# Autodesk Inventor assembly: 15inOwl
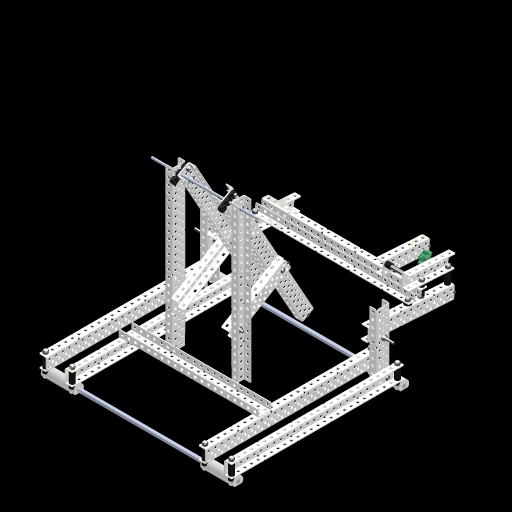
[picture p0: Inventor's stored thumbnail of the model, 512x512]
Saved by Autodesk Inventor 2024.1 (Build 281209000, 209)
## iProperties
Created: 2025-01-28
Part Number: 15inOwl
Document SubType Name: Assembly
Designer: Teddy
Author: Teddy
## Documents named in this file (38)
- C:\Users\Teddy\OneDrive\Desktop\VEX-CAD-Inventor-1.4.0\2024-25 VexGame\15inBotAub\15inOwl.iam
- C:\Users\Teddy\OneDrive\Desktop\VEX-CAD-Inventor-1.4.0\Structure\C Channel\Aluminum 1x2x1\Alu C 1x2x1x21.ipt
- C:\Users\Teddy\OneDrive\Desktop\VEX-CAD-Inventor-1.4.0\Structure\C Channel\Aluminum 1x2x1\Alu C 1x2x1x26.ipt
- C:\Users\Teddy\OneDrive\Desktop\AxleBar.ipt
- C:\Users\Teddy\OneDrive\Desktop\VEX-CAD-Inventor-1.4.0\Motion\Spacers\Spacer Nylon .375 OD\NSpacer .375 OD x .250.ipt
- C:\Users\Teddy\OneDrive\Desktop\VEX-CAD-Inventor-1.4.0\Motion\Spacers\Spacer Nylon .375 OD.ipt
- C:\Users\Teddy\OneDrive\Desktop\VEX-CAD-Inventor-1.4.0\Motion\Shaft HS\Shaft HS\Shaft HS 14.5 in.ipt
- C:\Users\Teddy\OneDrive\Desktop\VEX-CAD-Inventor-1.4.0\Motion\Shaft HS\Shaft HS.ipt
- C:\Users\Teddy\OneDrive\Desktop\VEX-CAD-Inventor-1.4.0\Structure\Hardware\Screw Steel - Star\SScrew Star Smooth 1.250.ipt
- C:\Users\Teddy\OneDrive\Desktop\VEX-CAD-Inventor-1.4.0\Structure\Hardware\Screw Steel - Star.ipt
- C:\Users\Teddy\OneDrive\Desktop\VEX-CAD-Inventor-1.4.0\Structure\Hardware\Screw Steel - Star\SScrew Star Smooth 1.750.ipt
- C:\Users\Teddy\OneDrive\Desktop\VEX-CAD-Inventor-1.4.0\Motion\Spacers\Spacer Nylon .375 OD\NSpacer .375 OD x .500.ipt
- C:\Users\Teddy\OneDrive\Desktop\VEX-CAD-Inventor-1.4.0\Motion\Spacers\Spacer Nylon .375 OD\NSpacer .375 OD x .375.ipt
- C:\Users\Teddy\OneDrive\Desktop\VEX-CAD-Inventor-1.4.0\Structure\Hardware\Nut Nylock.ipt
- C:\Users\Teddy\OneDrive\Desktop\VEX-CAD-Inventor-1.4.0\Structure\C Channel\Aluminum 1x2x1\Alu C 1x2x1x24.ipt
- C:\Users\Teddy\OneDrive\Desktop\VEX-CAD-Inventor-1.4.0\Structure\C Channel\Aluminum 1x2x1\Alu C 1x2x1x10.ipt
- C:\Users\Teddy\OneDrive\Desktop\VEX-CAD-Inventor-1.4.0\Structure\C Channel\Aluminum 1x2x1\Alu C 1x2x1x25.ipt
- C:\Users\Teddy\OneDrive\Desktop\VEX-CAD-Inventor-1.4.0\Motion\Spacers\Spacer Nylon .500 OD.ipt
- C:\Users\Teddy\OneDrive\Desktop\VEX-CAD-Inventor-1.4.0\Motion\Spacers\Spacer Nylon .500 OD\NSpacer White .500 OD x .375.ipt
- C:\Users\Teddy\OneDrive\Desktop\VEX-CAD-Inventor-1.4.0\Structure\Hardware\Screw Steel - Star\SScrew Star Smooth .750.ipt
- C:\Users\Teddy\OneDrive\Desktop\VEX-CAD-Inventor-1.4.0\Motion\Shaft LS\Shaft LS\Shaft LS 8.0.ipt
- C:\Users\Teddy\OneDrive\Desktop\VEX-CAD-Inventor-1.4.0\Motion\Shaft LS\Shaft LS.ipt
- C:\Users\Teddy\OneDrive\Desktop\VEX-CAD-Inventor-1.4.0\Motion\Shaft LS\Bearing Flat.ipt
- C:\Users\Teddy\OneDrive\Desktop\VEX-CAD-Inventor-1.4.0\Structure\Hardware\Screw Steel - Star\SScrew Star Smooth .625.ipt
- C:\Users\Teddy\OneDrive\Desktop\VEX-CAD-Inventor-1.4.0\Structure\Hardware\Screw Steel - Star\SScrew Star Smooth .500.ipt
- C:\Users\Teddy\OneDrive\Desktop\VEX-CAD-Inventor-1.4.0\Structure\Hardware\Screw Steel - Star\SScrew Star Smooth .375.ipt
- C:\Users\Teddy\OneDrive\Desktop\VEX-CAD-Inventor-1.4.0\Structure\C Channel\Aluminum 1x2x1\Alu C 1x2x1x13.ipt
- C:\Users\Teddy\OneDrive\Desktop\VEX-CAD-Inventor-1.4.0\Structure\Angle\Aluminum\1x1\Alu Angle 1x1x24.ipt
- C:\Users\Teddy\OneDrive\Desktop\VEX-CAD-Inventor-1.4.0\Structure\Hardware\Nut Keps.ipt
- C:\Users\Teddy\OneDrive\Desktop\VEX-CAD-Inventor-1.4.0\Motion\Spacers\Spacer Nylon .500 OD\NSpacer Black .500 OD x .125.ipt
- C:\Users\Teddy\OneDrive\Desktop\VEX-CAD-Inventor-1.4.0\Structure\C Channel\Aluminum 1x2x1\Alu C 1x2x1x7.ipt
- C:\Users\Teddy\OneDrive\Desktop\VEX-CAD-Inventor-1.4.0\Structure\Hardware\Screw Steel - Star\SScrew Star Smooth 1.500.ipt
- C:\Users\Teddy\OneDrive\Desktop\VEX-CAD-Inventor-1.4.0\Structure\Hardware\Screw Steel - Star\SScrew Star Smooth 2.250.ipt
- C:\Users\Teddy\OneDrive\Desktop\VEX-CAD-Inventor-1.4.0\Structure\Standoff.ipt
- C:\Users\Teddy\OneDrive\Desktop\VEX-CAD-Inventor-1.4.0\Structure\Standoff\Standoff 1.00.ipt
- C:\Users\Teddy\OneDrive\Desktop\VEX-CAD-Inventor-1.4.0\Motion\Sprockets\9P Sprocket.iam
- C:\Users\Teddy\OneDrive\Desktop\VEX-CAD-Inventor-1.4.0\Motion\Sprockets\9P Sprocket\9P 6T Sprocket, Square.iam
- C:\Users\Teddy\OneDrive\Desktop\VEX-CAD-Inventor-1.4.0\Motion\Spacers\Spacer Nylon .500 OD\NSpacer White .500 OD x .500.ipt
## Components (124 placed, 30 different names)
1. Alu C 1x2x1x21:1 — Insert:1, Insert:2, Insert:3, Insert:4, Insert:57, Insert:58
2. Alu C 1x2x1x26:1 — Insert:3, Insert:4, Insert:17, Insert:20, Insert:36, Insert:44, Insert:48, Insert:49
3. Alu C 1x2x1x26:2 — Insert:1, Insert:2, Insert:13, Insert:16, Insert:41, Insert:42, Insert:53, Insert:55
4. Alu C 1x2x1x26:3 — Insert:14, Insert:15, Insert:38, Insert:40, Insert:51, Insert:56, Insert:92, Insert:93, Insert:96, Insert:97
5. Alu C 1x2x1x26:4 — Insert:18, Insert:19, Insert:26, Insert:28, Insert:45, Insert:47, Insert:94, Insert:95, Insert:100, Insert:101
6. AxleBar:1 — Insert:9, Insert:10, Insert:22, Insert:34, Insert:35
7. AxleBar:2 — Insert:11, Insert:12, Insert:21, Insert:32, Insert:33
8. AxleBar:3 — Insert:7, Insert:8, Insert:23, Insert:29, Insert:30
9. AxleBar:4 — Insert:5, Insert:6, Insert:24, Insert:25, Insert:31
10. NSpacer .375 OD x .250:1 — Insert:5, Insert:18
11. NSpacer .375 OD x .250:2 — Insert:6, Insert:17
12. NSpacer .375 OD x .250:3 — Insert:7, Insert:16
13. NSpacer .375 OD x .250:4 — Insert:8, Insert:15
14. NSpacer .375 OD x .250:5 — Insert:12, Insert:14
15. NSpacer .375 OD x .250:6 — Insert:11, Insert:13
16. NSpacer .375 OD x .250:7 — Insert:10, Insert:20
17. NSpacer .375 OD x .250:8 — Insert:9, Insert:19
18. Shaft HS 14.5 in:1 — Insert:21, Insert:22
19. Shaft HS 14.5 in:2 — Insert:23, Insert:24
20. SScrew Star Smooth 1.750:1 — Insert:25
21. NSpacer .375 OD x .500:9 — Insert:26, Insert:27
22. NSpacer .375 OD x .375:10 — Insert:27
23. NSpacer .375 OD x .375:11 — Insert:50
24. NSpacer .375 OD x .375:12 — Insert:52
25. NSpacer .375 OD x .375:13 — Insert:54
26. NSpacer .375 OD x .375:14 — Insert:39
27. NSpacer .375 OD x .375:15 — Insert:43
28. NSpacer .375 OD x .375:16 — Insert:46
29. NSpacer .375 OD x .375:17 — Insert:37
30. NSpacer .375 OD x .500:18 — Insert:49, Insert:50
31. NSpacer .375 OD x .500:19 — Insert:53, Insert:54
32. NSpacer .375 OD x .500:20 — Insert:51, Insert:52
33. NSpacer .375 OD x .500:21 — Insert:38, Insert:39
34. NSpacer .375 OD x .500:22 — Insert:36, Insert:37
35. NSpacer .375 OD x .500:23 — Insert:45, Insert:46
36. NSpacer .375 OD x .500:24 — Insert:42, Insert:43
37. SScrew Star Smooth 1.750:2 — Insert:31
38. SScrew Star Smooth 1.750:3 — Insert:30
39. SScrew Star Smooth 1.750:4 — Insert:29
40. SScrew Star Smooth 1.750:5 — Insert:33
41. SScrew Star Smooth 1.750:6 — Insert:32
42. SScrew Star Smooth 1.750:7 — Insert:34
43. SScrew Star Smooth 1.750:8 — Insert:35
44. Nut Nylock:1 — Insert:47
45. Nut Nylock:2 — Insert:44
46. Nut Nylock:3 — Insert:56
47. Nut Nylock:4 — Insert:48
48. Nut Nylock:5 — Insert:55
49. Nut Nylock:6 — Insert:41
50. Nut Nylock:7 — Insert:40
51. Nut Nylock:8 — Insert:28
52. Alu C 1x2x1x24:1 — Insert:57, Insert:59, Insert:62, Insert:72, Insert:90
53. Alu C 1x2x1x24:2 — Insert:58, Insert:60, Insert:61, Insert:71, Insert:91
54. Alu C 1x2x1x10:1 — Insert:60, Insert:65, Insert:68, Insert:70, Insert:88
55. Alu C 1x2x1x10:2 — Insert:59, Insert:66, Insert:67, Insert:69, Insert:89
56. Alu C 1x2x1x25:1 — Insert:63, Insert:65, Insert:73, Insert:76, Insert:80, Insert:81
57. Alu C 1x2x1x25:2 — Insert:64, Insert:66, Insert:74, Insert:75, Insert:82, Insert:84, Insert:85
58. NSpacer .375 OD x .500:25 — Insert:61, Insert:63
59. NSpacer .375 OD x .500:26 — Insert:62, Insert:64
60. NSpacer White .500 OD x .375:1 — Insert:68
61. NSpacer White .500 OD x .375:2 — Insert:67
62. SScrew Star Smooth .750:9 — Insert:70
63. SScrew Star Smooth .750:10 — Insert:69
64. SScrew Star Smooth 1.250:11 — Insert:71
65. SScrew Star Smooth 1.250:12 — Insert:72
66. Nut Nylock:9 — Insert:74
67. Nut Nylock:10 — Insert:73
68. Nut Nylock:11 — Insert:75
69. Nut Nylock:12 — Insert:76
70. Bearing Flat:2 — Insert:80, Insert:81, Insert:83
71. SScrew Star Smooth .625:13 — Insert:83
72. Nut Nylock:13 — Insert:82
73. Bearing Flat:3 — Insert:84, Insert:85, Insert:86, Insert:87
74. SScrew Star Smooth .500:14 — Insert:86
75. Shaft LS 8.0:1 — Insert:87
76. SScrew Star Smooth .500:15 — Insert:88
77. SScrew Star Smooth .500:16 — Insert:89
78. Nut Nylock:14 — Insert:91
79. Nut Nylock:15 — Insert:90
80. Alu C 1x2x1x10:3 — Insert:92, Insert:93, Insert:98, Insert:99, Insert:135, Insert:138, Insert:141
81. Alu C 1x2x1x10:4 — Insert:94, Insert:95, Insert:102, Insert:103, Insert:139, Insert:140
82. SScrew Star Smooth .375:17 — Insert:97
83. SScrew Star Smooth .375:18 — Insert:96
84. Nut Nylock:16 — Insert:99
85. Nut Nylock:17 — Insert:98
86. Nut Nylock:18 — Insert:103
87. Nut Nylock:19 — Insert:102
88. SScrew Star Smooth .375:19 — Insert:100
89. SScrew Star Smooth .375:20 — Insert:101
90. Alu C 1x2x1x13:1 — Insert:104, Insert:107, Insert:114, Insert:117, Insert:118, Insert:119, Insert:120, Angle:1, Angle:2, Insert:137
91. Alu C 1x2x1x13:2 — Insert:121, Insert:124, Insert:125, Angle:3, Angle:4, Insert:135, Insert:136
92. Alu Angle 1x1x24:1 — Insert:108, Insert:109, Insert:126, Insert:127, Angle:1, Angle:3
93. Alu Angle 1x1x24:2 — Insert:106, Insert:110, Insert:123, Insert:128, Angle:2, Angle:4
94. Nut Keps:1 — Insert:104, Insert:105
95. Nut Keps:2 — Insert:121, Insert:122
96. NSpacer .375 OD x .500:27 — Insert:105, Insert:106
97. NSpacer Black .500 OD x .125:3 — Insert:107, Insert:108
98. Nut Nylock:20 — Insert:109
99. NSpacer .375 OD x .250:28 — Insert:110, Insert:111
100. Alu C 1x2x1x7:1 — Insert:111, Insert:112, Insert:113, Insert:130, Angle:5, Insert:134
101. Nut Nylock:21 — Insert:112
102. Nut Nylock:22 — Insert:113
103. Alu C 1x2x1x7:2 — Insert:129, Angle:5, Insert:133
104. NSpacer .375 OD x .500:29 — Insert:114, Insert:115
105. NSpacer .375 OD x .375:30 — Insert:115
106. NSpacer .375 OD x .500:31 — Insert:116, Insert:117
107. NSpacer .375 OD x .375:32 — Insert:116
108. SScrew Star Smooth 2.250:21 — Insert:118
109. SScrew Star Smooth 2.250:22 — Insert:119
110. SScrew Star Smooth 1.250:23 — Insert:120
111. NSpacer .375 OD x .500:33 — Insert:122, Insert:123
112. NSpacer Black .500 OD x .125:4 — Insert:124
113. SScrew Star Smooth 1.250:24 — Insert:125, Insert:126
114. Nut Nylock:23 — Insert:127
115. NSpacer .375 OD x .250:34 — Insert:128, Insert:129
116. Standoff 1.00:1 — Insert:130, Insert:132
117. NSpacer .375 OD x .375:35 — Insert:132, Insert:133
118. 9P 6T Sprocket, Square:1 [sub-assembly] — Insert:134
119. SScrew Star Smooth 1.500:25 — Insert:136
120. SScrew Star Smooth 1.500:26 — Insert:137
121. Nut Nylock:24 — Insert:139
122. Nut Nylock:25 — Insert:138
123. NSpacer White .500 OD x .500:5 — Insert:140
124. NSpacer White .500 OD x .500:6 — Insert:141
## Relationships (142: Insert 137, Angle 5)
- Insert:1: Alu C 1x2x1x21:1 ↔ Alu C 1x2x1x26:2
- Insert:2: Alu C 1x2x1x21:1 ↔ Alu C 1x2x1x26:2
- Insert:3: Alu C 1x2x1x21:1 ↔ Alu C 1x2x1x26:1
- Insert:4: Alu C 1x2x1x21:1 ↔ Alu C 1x2x1x26:1
- Insert:5: AxleBar:4 ↔ NSpacer .375 OD x .250:1
- Insert:6: AxleBar:4 ↔ NSpacer .375 OD x .250:2
- Insert:7: AxleBar:3 ↔ NSpacer .375 OD x .250:3
- Insert:8: AxleBar:3 ↔ NSpacer .375 OD x .250:4
- Insert:9: AxleBar:1 ↔ NSpacer .375 OD x .250:8
- Insert:10: AxleBar:1 ↔ NSpacer .375 OD x .250:7
- Insert:11: AxleBar:2 ↔ NSpacer .375 OD x .250:6
- Insert:12: AxleBar:2 ↔ NSpacer .375 OD x .250:5
- Insert:13: Alu C 1x2x1x26:2 ↔ NSpacer .375 OD x .250:6
- Insert:14: Alu C 1x2x1x26:3 ↔ NSpacer .375 OD x .250:5
- Insert:15: Alu C 1x2x1x26:3 ↔ NSpacer .375 OD x .250:4
- Insert:16: Alu C 1x2x1x26:2 ↔ NSpacer .375 OD x .250:3
- Insert:17: Alu C 1x2x1x26:1 ↔ NSpacer .375 OD x .250:2
- Insert:18: Alu C 1x2x1x26:4 ↔ NSpacer .375 OD x .250:1
- Insert:19: Alu C 1x2x1x26:4 ↔ NSpacer .375 OD x .250:8
- Insert:20: Alu C 1x2x1x26:1 ↔ NSpacer .375 OD x .250:7
- Insert:21: AxleBar:2 ↔ Shaft HS 14.5 in:1
- Insert:22: AxleBar:1 ↔ Shaft HS 14.5 in:1
- Insert:23: AxleBar:3 ↔ Shaft HS 14.5 in:2
- Insert:24: AxleBar:4 ↔ Shaft HS 14.5 in:2
- Insert:25: AxleBar:4 ↔ SScrew Star Smooth 1.750:1
- Insert:26: Alu C 1x2x1x26:4 ↔ NSpacer .375 OD x .500:9
- Insert:27: NSpacer .375 OD x .500:9 ↔ NSpacer .375 OD x .375:10
- Insert:28: Alu C 1x2x1x26:4 ↔ Nut Nylock:8
- Insert:29: AxleBar:3 ↔ SScrew Star Smooth 1.750:4
- Insert:30: AxleBar:3 ↔ SScrew Star Smooth 1.750:3
- Insert:31: AxleBar:4 ↔ SScrew Star Smooth 1.750:2
- Insert:32: AxleBar:2 ↔ SScrew Star Smooth 1.750:6
- Insert:33: AxleBar:2 ↔ SScrew Star Smooth 1.750:5
- Insert:34: AxleBar:1 ↔ SScrew Star Smooth 1.750:7
- Insert:35: AxleBar:1 ↔ SScrew Star Smooth 1.750:8
- Insert:36: Alu C 1x2x1x26:1 ↔ NSpacer .375 OD x .500:22
- Insert:37: NSpacer .375 OD x .375:17 ↔ NSpacer .375 OD x .500:22
- Insert:38: Alu C 1x2x1x26:3 ↔ NSpacer .375 OD x .500:21
- Insert:39: NSpacer .375 OD x .375:14 ↔ NSpacer .375 OD x .500:21
- Insert:40: Alu C 1x2x1x26:3 ↔ Nut Nylock:7
- Insert:41: Alu C 1x2x1x26:2 ↔ Nut Nylock:6
- Insert:42: Alu C 1x2x1x26:2 ↔ NSpacer .375 OD x .500:24
- Insert:43: NSpacer .375 OD x .375:15 ↔ NSpacer .375 OD x .500:24
- Insert:44: Alu C 1x2x1x26:1 ↔ Nut Nylock:2
- Insert:45: Alu C 1x2x1x26:4 ↔ NSpacer .375 OD x .500:23
- Insert:46: NSpacer .375 OD x .375:16 ↔ NSpacer .375 OD x .500:23
- Insert:47: Alu C 1x2x1x26:4 ↔ Nut Nylock:1
- Insert:48: Alu C 1x2x1x26:1 ↔ Nut Nylock:4
- Insert:49: Alu C 1x2x1x26:1 ↔ NSpacer .375 OD x .500:18
- Insert:50: NSpacer .375 OD x .375:11 ↔ NSpacer .375 OD x .500:18
- Insert:51: Alu C 1x2x1x26:3 ↔ NSpacer .375 OD x .500:20
- Insert:52: NSpacer .375 OD x .375:12 ↔ NSpacer .375 OD x .500:20
- Insert:53: Alu C 1x2x1x26:2 ↔ NSpacer .375 OD x .500:19
- Insert:54: NSpacer .375 OD x .375:13 ↔ NSpacer .375 OD x .500:19
- Insert:55: Alu C 1x2x1x26:2 ↔ Nut Nylock:5
- Insert:56: Alu C 1x2x1x26:3 ↔ Nut Nylock:3
- Insert:57: Alu C 1x2x1x21:1 ↔ Alu C 1x2x1x24:1
- Insert:58: Alu C 1x2x1x21:1 ↔ Alu C 1x2x1x24:2
- Insert:59: Alu C 1x2x1x24:1 ↔ Alu C 1x2x1x10:2
- Insert:60: Alu C 1x2x1x24:2 ↔ Alu C 1x2x1x10:1
- Insert:61: Alu C 1x2x1x24:2 ↔ NSpacer .375 OD x .500:25
- Insert:62: Alu C 1x2x1x24:1 ↔ NSpacer .375 OD x .500:26
- Insert:63: Alu C 1x2x1x25:1 ↔ NSpacer .375 OD x .500:25
- Insert:64: Alu C 1x2x1x25:2 ↔ NSpacer .375 OD x .500:26
- Insert:65: Alu C 1x2x1x10:1 ↔ Alu C 1x2x1x25:1
- Insert:66: Alu C 1x2x1x10:2 ↔ Alu C 1x2x1x25:2
- Insert:67: Alu C 1x2x1x10:2 ↔ NSpacer White .500 OD x .375:2
- Insert:68: Alu C 1x2x1x10:1 ↔ NSpacer White .500 OD x .375:1
- Insert:69: Alu C 1x2x1x10:2 ↔ SScrew Star Smooth .750:10
- Insert:70: Alu C 1x2x1x10:1 ↔ SScrew Star Smooth .750:9
- Insert:71: Alu C 1x2x1x24:2 ↔ SScrew Star Smooth 1.250:11
- Insert:72: Alu C 1x2x1x24:1 ↔ SScrew Star Smooth 1.250:12
- Insert:73: Alu C 1x2x1x25:1 ↔ Nut Nylock:10
- Insert:74: Alu C 1x2x1x25:2 ↔ Nut Nylock:9
- Insert:75: Alu C 1x2x1x25:2 ↔ Nut Nylock:11
- Insert:76: Alu C 1x2x1x25:1 ↔ Nut Nylock:12
- Insert:80: Alu C 1x2x1x25:1 ↔ Bearing Flat:2
- Insert:81: Alu C 1x2x1x25:1 ↔ Bearing Flat:2
- Insert:82: Alu C 1x2x1x25:2 ↔ Nut Nylock:13
- Insert:83: Bearing Flat:2 ↔ SScrew Star Smooth .625:13
- Insert:84: Alu C 1x2x1x25:2 ↔ Bearing Flat:3
- Insert:85: Alu C 1x2x1x25:2 ↔ Bearing Flat:3
- Insert:86: Bearing Flat:3 ↔ SScrew Star Smooth .500:14
- Insert:87 (-50.8 mm): Bearing Flat:3 ↔ Shaft LS 8.0:1
- Insert:88: Alu C 1x2x1x10:1 ↔ SScrew Star Smooth .500:15
- Insert:89: Alu C 1x2x1x10:2 ↔ SScrew Star Smooth .500:16
- Insert:90: Alu C 1x2x1x24:1 ↔ Nut Nylock:15
- Insert:91: Alu C 1x2x1x24:2 ↔ Nut Nylock:14
- Insert:92: Alu C 1x2x1x26:3 ↔ Alu C 1x2x1x10:3
- Insert:93: Alu C 1x2x1x26:3 ↔ Alu C 1x2x1x10:3
- Insert:94: Alu C 1x2x1x26:4 ↔ Alu C 1x2x1x10:4
- Insert:95: Alu C 1x2x1x26:4 ↔ Alu C 1x2x1x10:4
- Insert:96: Alu C 1x2x1x26:3 ↔ SScrew Star Smooth .375:18
- Insert:97: Alu C 1x2x1x26:3 ↔ SScrew Star Smooth .375:17
- Insert:98: Alu C 1x2x1x10:3 ↔ Nut Nylock:17
- Insert:99: Alu C 1x2x1x10:3 ↔ Nut Nylock:16
- Insert:100: Alu C 1x2x1x26:4 ↔ SScrew Star Smooth .375:19
- Insert:101: Alu C 1x2x1x26:4 ↔ SScrew Star Smooth .375:20
- Insert:102: Alu C 1x2x1x10:4 ↔ Nut Nylock:19
- Insert:103: Alu C 1x2x1x10:4 ↔ Nut Nylock:18
- Insert:104: Alu C 1x2x1x13:1 ↔ Nut Keps:1
- Insert:105: Nut Keps:1 ↔ NSpacer .375 OD x .500:27
- Insert:106: Alu Angle 1x1x24:2 ↔ NSpacer .375 OD x .500:27
- Insert:107: Alu C 1x2x1x13:1 ↔ NSpacer Black .500 OD x .125:3
- Insert:108: Alu Angle 1x1x24:1 ↔ NSpacer Black .500 OD x .125:3
- Insert:109: Alu Angle 1x1x24:1 ↔ Nut Nylock:20
- Insert:110: Alu Angle 1x1x24:2 ↔ NSpacer .375 OD x .250:28
- Insert:111: NSpacer .375 OD x .250:28 ↔ Alu C 1x2x1x7:1
- Insert:112: Alu C 1x2x1x7:1 ↔ Nut Nylock:21
- Insert:113: Alu C 1x2x1x7:1 ↔ Nut Nylock:22
- Insert:114: Alu C 1x2x1x13:1 ↔ NSpacer .375 OD x .500:29
- Insert:115: NSpacer .375 OD x .500:29 ↔ NSpacer .375 OD x .375:30
- Insert:116: NSpacer .375 OD x .500:31 ↔ NSpacer .375 OD x .375:32
- Insert:117: Alu C 1x2x1x13:1 ↔ NSpacer .375 OD x .500:31
- Insert:118: Alu C 1x2x1x13:1 ↔ SScrew Star Smooth 2.250:21
- Insert:119: Alu C 1x2x1x13:1 ↔ SScrew Star Smooth 2.250:22
- Insert:120: Alu C 1x2x1x13:1 ↔ SScrew Star Smooth 1.250:23
- Insert:121: Alu C 1x2x1x13:2 ↔ Nut Keps:2
- Insert:122: Nut Keps:2 ↔ NSpacer .375 OD x .500:33
- Insert:123: Alu Angle 1x1x24:2 ↔ NSpacer .375 OD x .500:33
- Insert:124: Alu C 1x2x1x13:2 ↔ NSpacer Black .500 OD x .125:4
- Insert:125: Alu C 1x2x1x13:2 ↔ SScrew Star Smooth 1.250:24
- Insert:126: Alu Angle 1x1x24:1 ↔ SScrew Star Smooth 1.250:24
- Insert:127: Alu Angle 1x1x24:1 ↔ Nut Nylock:23
- Insert:128: Alu Angle 1x1x24:2 ↔ NSpacer .375 OD x .250:34
- Insert:129: Alu C 1x2x1x7:2 ↔ NSpacer .375 OD x .250:34
- Angle:1 (180 deg): Alu C 1x2x1x13:1 ↔ Alu Angle 1x1x24:1
- Angle:2 (180 deg): Alu C 1x2x1x13:1 ↔ Alu Angle 1x1x24:2
- Angle:3 (180 deg): Alu C 1x2x1x13:2 ↔ Alu Angle 1x1x24:1
- Angle:4 (180 deg): Alu C 1x2x1x13:2 ↔ Alu Angle 1x1x24:2
- Insert:130: Alu C 1x2x1x7:1 ↔ Standoff 1.00:1
- Insert:132: Standoff 1.00:1 ↔ NSpacer .375 OD x .375:35
- Angle:5 (0 deg): Alu C 1x2x1x7:1 ↔ Alu C 1x2x1x7:2
- Insert:133: Alu C 1x2x1x7:2 ↔ NSpacer .375 OD x .375:35
- Insert:134 (11.43 mm): Alu C 1x2x1x7:1 ↔ 9P 6T Sprocket, Square:1
- Insert:135 (13.97 mm): Alu C 1x2x1x10:3 ↔ Alu C 1x2x1x13:2
- Insert:136: Alu C 1x2x1x13:2 ↔ SScrew Star Smooth 1.500:25
- Insert:137: Alu C 1x2x1x13:1 ↔ SScrew Star Smooth 1.500:26
- Insert:138: Alu C 1x2x1x10:3 ↔ Nut Nylock:25
- Insert:139: Alu C 1x2x1x10:4 ↔ Nut Nylock:24
- Insert:140: Alu C 1x2x1x10:4 ↔ NSpacer White .500 OD x .500:5
- Insert:141: Alu C 1x2x1x10:3 ↔ NSpacer White .500 OD x .500:6
